# Autodesk Inventor assembly: Assembly1
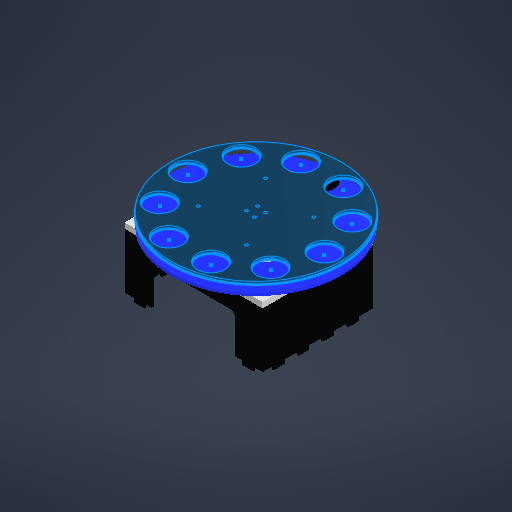
[picture p0: Inventor's stored thumbnail of the model, 512x512]
Saved by Autodesk Inventor 2027.1 (Build 311270010, 270A)
## iProperties
Created: 2026-09-28
Part Number: Assembly1
Document SubType Name: Assembly
Designer: daniel
Author: daniel
## Documents named in this file (8)
- E:\Apps\AutodeskInventor\University\MCT333_Design_of_Mechatronics_Systems_1\CAD\FEED and Sorting\Assembly1.iam
- E:\Apps\AutodeskInventor\University\MCT333_Design_of_Mechatronics_Systems_1\CAD\FEED and Sorting\Part2.ipt
- E:\Apps\AutodeskInventor\University\MCT333_Design_of_Mechatronics_Systems_1\CAD\FEED and Sorting\Part1.ipt
- E:\Apps\AutodeskInventor\University\MCT333_Design_of_Mechatronics_Systems_1\CAD\off_the_shelf_components\standard-servo-motor-black-1.snapshot.7\Assem1\Assem1.iam
- E:\Apps\AutodeskInventor\University\MCT333_Design_of_Mechatronics_Systems_1\CAD\FEED and Sorting\Part67.ipt
- C:\Users\SDS Scholar\Documents\Inventor\Content Center Files\R2027\en-US\GB_T 301-1995(51000)\Rolling bearing 51109 GB_T 301-1995.ipt
- E:\Apps\AutodeskInventor\University\MCT333_Design_of_Mechatronics_Systems_1\CAD\FEED and Sorting\Part69.ipt
- E:\Apps\AutodeskInventor\University\MCT333_Design_of_Mechatronics_Systems_1\CAD\FEED and Sorting\box\MagazineBox.iam
## Components (8 placed, 7 different names)
1. MagazineBox:1 [sub-assembly] — Mate:2, Mate:3, Mate:4, Flush:2, Mate:9, Mate:10, Mate:11, Flush:3
2. Part2:1 — Mate:13, Mate:14, Mate:15, Mate:16
3. Part1:1 — Mate:2, Mate:3, Mate:5, Mate:6, Mate:7, Mate:8, Mate:12
4. Assem1:1 [sub-assembly] — Mate:9, Mate:10, Mate:11, Mate:16
5. Part67:1 — Mate:4, Flush:2, Mate:5, Flush:3
6. Rolling bearing GB/T 301-1995 Type 51000 51109:1 — Mate:12, Tangent:1, Tangent:2
7. Part69:1 — Mate:13, Mate:14, Mate:15, Tangent:2
8. Part69:2 — Mate:6, Mate:7, Mate:8, Tangent:1
## Relationships (19: Mate 15, Flush 2, Tangent 2)
- Mate:2: MagazineBox:1 ↔ Part1:1
- Mate:3: MagazineBox:1 ↔ Part1:1
- Mate:4: MagazineBox:1 ↔ Part67:1
- Flush:2: MagazineBox:1 ↔ Part67:1
- Mate:5: Part1:1 ↔ Part67:1
- Mate:6: Part1:1 ↔ Part69:2
- Mate:7: Part1:1 ↔ Part69:2
- Mate:8: Part1:1 ↔ Part69:2
- Mate:9: MagazineBox:1 ↔ Assem1:1
- Mate:10: MagazineBox:1 ↔ Assem1:1
- Mate:11: MagazineBox:1 ↔ Assem1:1
- Mate:12: Part1:1 ↔ Rolling bearing GB/T 301-1995 Type 51000 51109:1
- Tangent:1: Rolling bearing GB/T 301-1995 Type 51000 51109:1 ↔ Part69:2
- Mate:13: Part2:1 ↔ Part69:1
- Mate:14: Part2:1 ↔ Part69:1
- Mate:15: Part2:1 ↔ Part69:1
- Tangent:2: Rolling bearing GB/T 301-1995 Type 51000 51109:1 ↔ Part69:1
- Mate:16: Part2:1 ↔ Assem1:1
- Flush:3: MagazineBox:1 ↔ Part67:1
